# Autodesk Inventor assembly: Solenoid
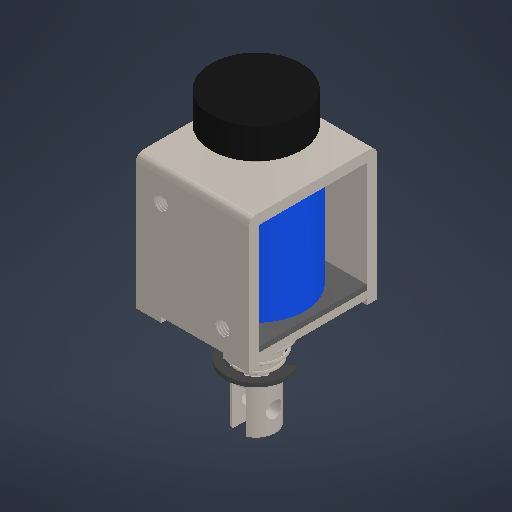
[picture p0: Inventor's stored thumbnail of the model, 512x512]
Saved by Autodesk Inventor 2026.1 (Build 301233020, 233B)
## iProperties
Created: 2025-11-08
Part Number: Solenoid
Document SubType Name: Assembly
Designer: Bahaa
Author: Bahaa
## Documents named in this file (4)
- C:\Users\Bahaa\Nextcloud2\CAD\25-26\Solenoid.iam
- C:\Users\Bahaa\Nextcloud2\CAD\25-26\Solenoid JF-0826B\Solenoid JF-0826B\Solenoid JF-0826B.ipt
- C:\Users\Bahaa\Nextcloud2\CAD\25-26\Solenoid Shield.ipt
- C:\Users\Bahaa\Documents\Inventor\Content Center Files\R2026\en-US\DIN 985\DIN 985 - M3.ipt
## Components (3 placed, 3 different names)
1. Solenoid JF-0826B:1 — Mate:4, Mate:5
2. Solenoid Shield:1 — Mate:1, Mate:2, Mate:5, Mate:6
3. DIN 985 - replaced by DIN EN ISO 10511 M3:1 — Mate:1, Mate:2, Mate:4, Mate:6
## Relationships (5: Mate 5)
- Mate:1: Solenoid Shield:1 ↔ DIN 985 - replaced by DIN EN ISO 10511 M3:1
- Mate:2: Solenoid Shield:1 ↔ DIN 985 - replaced by DIN EN ISO 10511 M3:1
- Mate:4: Solenoid JF-0826B:1 ↔ DIN 985 - replaced by DIN EN ISO 10511 M3:1
- Mate:5: Solenoid JF-0826B:1 ↔ Solenoid Shield:1
- Mate:6: Solenoid Shield:1 ↔ DIN 985 - replaced by DIN EN ISO 10511 M3:1
